# Autodesk Inventor assembly: HandLeft
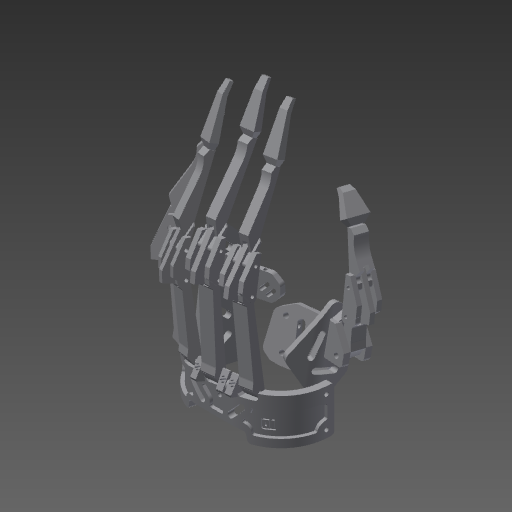
[picture p0: Inventor's stored thumbnail of the model, 512x512]
Saved by Autodesk Inventor 2020 (Build 240168000, 168)
## iProperties
Created: 2016-10-02
Part Number: HandLeft
Document SubType Name: Assembly
Designer: Val
Author: Val
## Documents named in this file (27)
- C:\Users\valer\Desktop\elysium-max-exoskeleton\src\Assemblies\HandLeft.iam
- C:\Users\valer\Desktop\elysium-max-exoskeleton\src\HandRibLeft.ipt
- C:\Users\valer\Desktop\elysium-max-exoskeleton\src\HandShockPlateLeft.ipt
- C:\Users\valer\Desktop\elysium-max-exoskeleton\src\ThumbShockPlateLeft.ipt
- C:\Users\valer\Desktop\elysium-max-exoskeleton\src\DistPhalangeThumb.ipt
- C:\Users\valer\Desktop\elysium-max-exoskeleton\src\MetacarpusThumb.ipt
- C:\Users\valer\Desktop\elysium-max-exoskeleton\src\ProxPhalangeThumb.ipt
- C:\Users\valer\Desktop\elysium-max-exoskeleton\src\ThumbMount.ipt
- C:\Users\valer\Desktop\elysium-max-exoskeleton\src\DistPhalangeIndex.ipt
- C:\Users\valer\Desktop\elysium-max-exoskeleton\src\DistPhalangeMiddle.ipt
- C:\Users\valer\Desktop\elysium-max-exoskeleton\src\DistPhalangePinky.ipt
- C:\Users\valer\Desktop\elysium-max-exoskeleton\src\DistPhalangeRing.ipt
- C:\Users\valer\Desktop\elysium-max-exoskeleton\src\ProxPhalangeIndex.ipt
- C:\Users\valer\Desktop\elysium-max-exoskeleton\src\ProxPhalangeMiddle.ipt
- C:\Users\valer\Desktop\elysium-max-exoskeleton\src\ProxPhalangePinky.ipt
- C:\Users\valer\Desktop\elysium-max-exoskeleton\src\ProxPhalangeRing.ipt
- C:\Users\valer\Desktop\elysium-max-exoskeleton\src\MetacarpusIndex.ipt
- C:\Users\valer\Desktop\elysium-max-exoskeleton\src\MetacarpusMiddle.ipt
- C:\Users\valer\Desktop\elysium-max-exoskeleton\src\MetacarpusPinky.ipt
- C:\Users\valer\Desktop\elysium-max-exoskeleton\src\MetacarpusRing.ipt
- C:\Users\valer\Desktop\elysium-max-exoskeleton\src\Knuckle.ipt
- C:\Users\valer\Desktop\elysium-max-exoskeleton\src\KnuckleSide.ipt
- C:\Users\valer\Desktop\elysium-max-exoskeleton\src\IndexRouter.ipt
- C:\Users\valer\Desktop\elysium-max-exoskeleton\src\MiddleRouter.ipt
- C:\Users\valer\Desktop\elysium-max-exoskeleton\src\PinkyRouter.ipt
- C:\Users\valer\Desktop\elysium-max-exoskeleton\src\RingRouter.ipt
- C:\Users\valer\Desktop\elysium-max-exoskeleton\src\ThumbRouter.ipt
## Components (39 placed, 26 different names)
1. HandRibLeft:1 — Mate:1, Mate:2
2. HandShockPlateLeft:1 — Mate:1, Mate:2, Mate:3, Mate:4, Mate:15, Angle:2, Mate:28, Angle:3, Mate:48, Angle:4, Mate:61, Angle:5
3. ThumbShockPlateLeft:1 — Mate:3, Mate:4, Mate:5, Mate:6, Angle:1
4. DistPhalangeThumb:1 — Mate:9, Mate:10
5. MetacarpusThumb:1 — Mate:7, Mate:8, Mate:11, Mate:12, Mate:29, Mate:30, Mate:34, Mate:35
6. ProxPhalangeThumb:1 — Mate:9, Mate:10, Mate:13, Mate:14, Mate:31, Mate:36
7. ThumbMount:1 — Mate:5, Mate:6, Angle:1, Mate:7, Mate:8
8. DistPhalangeIndex:1 — Mate:23, Mate:46
9. DistPhalangeMiddle:1 — Mate:45, Mate:47
10. DistPhalangePinky:1 — Mate:66, Mate:67
11. DistPhalangeRing:1 — Mate:53, Mate:54
12. ProxPhalangeIndex:1 — Mate:18, Mate:19, Mate:22, Mate:23, Mate:27, Mate:46
13. ProxPhalangeMiddle:1 — Mate:37, Mate:38, Mate:41, Mate:44, Mate:45, Mate:47
14. ProxPhalangePinky:1 — Mate:64, Mate:65, Mate:66, Mate:67, Mate:70, Mate:73
15. ProxPhalangeRing:1 — Mate:51, Mate:52, Mate:53, Mate:54, Mate:57, Mate:60
16. MetacarpusIndex:1 — Mate:15, Angle:2, Mate:16, Mate:17, Mate:20, Mate:21, Mate:25, Mate:26
17. MetacarpusMiddle:1 — Mate:28, Angle:3, Mate:32, Mate:33, Mate:39, Mate:40, Mate:42, Mate:43
18. MetacarpusPinky:1 — Mate:61, Angle:5, Mate:62, Mate:63, Mate:68, Mate:69, Mate:71, Mate:72
19. MetacarpusRing:1 — Mate:48, Angle:4, Mate:49, Mate:50, Mate:55, Mate:56, Mate:58, Mate:59
20. Knuckle:1 — Mate:11, Mate:12, Mate:13, Mate:14
21. Knuckle:2 — Mate:16, Mate:17, Mate:18, Mate:19
22. Knuckle:3 — Mate:32, Mate:33, Mate:37, Mate:38
23. Knuckle:4 — Mate:49, Mate:50, Mate:51, Mate:52
24. Knuckle:5 — Mate:62, Mate:63, Mate:64, Mate:65
25. KnuckleSide:1 — Mate:42, Mate:43, Mate:44
26. KnuckleSide:2 — Mate:39, Mate:40, Mate:41
27. KnuckleSide:3 — Mate:55, Mate:56, Mate:57
28. KnuckleSide:4 — Mate:58, Mate:59, Mate:60
29. KnuckleSide:5 — Mate:29, Mate:30, Mate:31
30. KnuckleSide:6 — Mate:34, Mate:35, Mate:36
31. KnuckleSide:7 — Mate:68, Mate:69, Mate:70
32. KnuckleSide:8 — Mate:71, Mate:72, Mate:73
33. KnuckleSide:9 — Mate:25, Mate:26, Mate:27
34. KnuckleSide:10 — Mate:20, Mate:21, Mate:22
35. IndexRouter:1
36. MiddleRouter:1
37. PinkyRouter:1
38. RingRouter:1
39. ThumbRouter:1
## Relationships (77: Mate 72, Angle 5)
- Mate:1: HandRibLeft:1 ↔ HandShockPlateLeft:1
- Mate:2: HandRibLeft:1 ↔ HandShockPlateLeft:1
- Mate:3: HandShockPlateLeft:1 ↔ ThumbShockPlateLeft:1
- Mate:4: HandShockPlateLeft:1 ↔ ThumbShockPlateLeft:1
- Mate:5: ThumbShockPlateLeft:1 ↔ ThumbMount:1
- Mate:6: ThumbShockPlateLeft:1 ↔ ThumbMount:1
- Angle:1 (0 deg): ThumbShockPlateLeft:1 ↔ ThumbMount:1
- Mate:7: MetacarpusThumb:1 ↔ ThumbMount:1
- Mate:8: MetacarpusThumb:1 ↔ ThumbMount:1
- Mate:9: DistPhalangeThumb:1 ↔ ProxPhalangeThumb:1
- Mate:10: DistPhalangeThumb:1 ↔ ProxPhalangeThumb:1
- Mate:11: MetacarpusThumb:1 ↔ Knuckle:1
- Mate:12: MetacarpusThumb:1 ↔ Knuckle:1
- Mate:13: ProxPhalangeThumb:1 ↔ Knuckle:1
- Mate:14: ProxPhalangeThumb:1 ↔ Knuckle:1
- Mate:15: HandShockPlateLeft:1 ↔ MetacarpusIndex:1
- Angle:2 (6 deg): HandShockPlateLeft:1 ↔ MetacarpusIndex:1
- Mate:16: MetacarpusIndex:1 ↔ Knuckle:2
- Mate:17: MetacarpusIndex:1 ↔ Knuckle:2
- Mate:18: ProxPhalangeIndex:1 ↔ Knuckle:2
- Mate:19: ProxPhalangeIndex:1 ↔ Knuckle:2
- Mate:20: MetacarpusIndex:1 ↔ KnuckleSide:10
- Mate:21: MetacarpusIndex:1 ↔ KnuckleSide:10
- Mate:22: ProxPhalangeIndex:1 ↔ KnuckleSide:10
- Mate:23: DistPhalangeIndex:1 ↔ ProxPhalangeIndex:1
- Mate:25: MetacarpusIndex:1 ↔ KnuckleSide:9
- Mate:26: MetacarpusIndex:1 ↔ KnuckleSide:9
- Mate:27: ProxPhalangeIndex:1 ↔ KnuckleSide:9
- Mate:28: HandShockPlateLeft:1 ↔ MetacarpusMiddle:1
- Angle:3 (0 deg): HandShockPlateLeft:1 ↔ MetacarpusMiddle:1
- Mate:29: MetacarpusThumb:1 ↔ KnuckleSide:5
- Mate:30: MetacarpusThumb:1 ↔ KnuckleSide:5
- Mate:31: ProxPhalangeThumb:1 ↔ KnuckleSide:5
- Mate:32: MetacarpusMiddle:1 ↔ Knuckle:3
- Mate:33: MetacarpusMiddle:1 ↔ Knuckle:3
- Mate:34: MetacarpusThumb:1 ↔ KnuckleSide:6
- Mate:35: MetacarpusThumb:1 ↔ KnuckleSide:6
- Mate:36: ProxPhalangeThumb:1 ↔ KnuckleSide:6
- Mate:37: ProxPhalangeMiddle:1 ↔ Knuckle:3
- Mate:38: ProxPhalangeMiddle:1 ↔ Knuckle:3
- Mate:39: MetacarpusMiddle:1 ↔ KnuckleSide:2
- Mate:40: MetacarpusMiddle:1 ↔ KnuckleSide:2
- Mate:41: ProxPhalangeMiddle:1 ↔ KnuckleSide:2
- Mate:42: MetacarpusMiddle:1 ↔ KnuckleSide:1
- Mate:43: MetacarpusMiddle:1 ↔ KnuckleSide:1
- Mate:44: ProxPhalangeMiddle:1 ↔ KnuckleSide:1
- Mate:45: DistPhalangeMiddle:1 ↔ ProxPhalangeMiddle:1
- Mate:46: DistPhalangeIndex:1 ↔ ProxPhalangeIndex:1
- Mate:47: DistPhalangeMiddle:1 ↔ ProxPhalangeMiddle:1
- Mate:48: HandShockPlateLeft:1 ↔ MetacarpusRing:1
- Angle:4 (0 deg): HandShockPlateLeft:1 ↔ MetacarpusRing:1
- Mate:49: MetacarpusRing:1 ↔ Knuckle:4
- Mate:50: MetacarpusRing:1 ↔ Knuckle:4
- Mate:51: ProxPhalangeRing:1 ↔ Knuckle:4
- Mate:52: ProxPhalangeRing:1 ↔ Knuckle:4
- Mate:53: DistPhalangeRing:1 ↔ ProxPhalangeRing:1
- Mate:54: DistPhalangeRing:1 ↔ ProxPhalangeRing:1
- Mate:55: MetacarpusRing:1 ↔ KnuckleSide:3
- Mate:56: MetacarpusRing:1 ↔ KnuckleSide:3
- Mate:57: ProxPhalangeRing:1 ↔ KnuckleSide:3
- Mate:58: MetacarpusRing:1 ↔ KnuckleSide:4
- Mate:59: MetacarpusRing:1 ↔ KnuckleSide:4
- Mate:60: ProxPhalangeRing:1 ↔ KnuckleSide:4
- Mate:61: HandShockPlateLeft:1 ↔ MetacarpusPinky:1
- Angle:5 (0 deg): HandShockPlateLeft:1 ↔ MetacarpusPinky:1
- Mate:62: MetacarpusPinky:1 ↔ Knuckle:5
- Mate:63: MetacarpusPinky:1 ↔ Knuckle:5
- Mate:64: ProxPhalangePinky:1 ↔ Knuckle:5
- Mate:65: ProxPhalangePinky:1 ↔ Knuckle:5
- Mate:66: DistPhalangePinky:1 ↔ ProxPhalangePinky:1
- Mate:67: DistPhalangePinky:1 ↔ ProxPhalangePinky:1
- Mate:68: MetacarpusPinky:1 ↔ KnuckleSide:7
- Mate:69: MetacarpusPinky:1 ↔ KnuckleSide:7
- Mate:70: ProxPhalangePinky:1 ↔ KnuckleSide:7
- Mate:71: MetacarpusPinky:1 ↔ KnuckleSide:8
- Mate:72: MetacarpusPinky:1 ↔ KnuckleSide:8
- Mate:73: ProxPhalangePinky:1 ↔ KnuckleSide:8
